# Autodesk Inventor assembly: handle
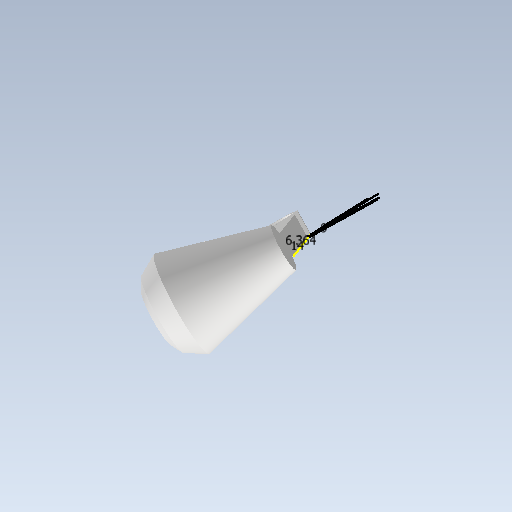
[picture p0: Inventor's stored thumbnail of the model, 512x512]
Saved by Autodesk Inventor 2021 (Build 250183000, 183)
## iProperties
Created: 2021-06-09
Part Number: handle
Document SubType Name: Assembly
Designer: teh18
Author: teh18
## Documents named in this file (4)
- C:\Users\teh18\OneDrive\BVE Controller\r68-bve-mascon\handle\handle.iam
- C:\Users\teh18\OneDrive\BVE Controller\r68-bve-mascon\handle\metal.ipt
- C:\Users\teh18\OneDrive\BVE Controller\r68-bve-mascon\handle\free-rotating sheath.ipt
- C:\Users\teh18\OneDrive\BVE Controller\r68-bve-mascon\handle\sheath cap.ipt
## Components (3 placed, 3 different names)
1. metal:1 — Rotational:1
2. free-rotating sheath:1 — Mate:6, Flush:1, Rotational:1
3. sheath cap:1 — Mate:6, Flush:1
## Relationships (3: Mate 1, Flush 1, RevoluteJoint 1)
- Mate:6: free-rotating sheath:1 ↔ sheath cap:1
- Flush:1: free-rotating sheath:1 ↔ sheath cap:1
- Rotational:1 [RevoluteJoint]: metal:1 ↔ free-rotating sheath:1
